# Autodesk Inventor assembly: szachy main
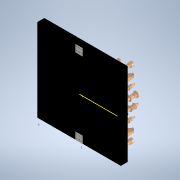
[picture p0: Inventor's stored thumbnail of the model, 180x180]
Saved by Autodesk Inventor 2021 (Build 250183000, 183)
## iProperties
Created: 2021-01-12
Part Number: szachy main
Document SubType Name: Assembly
Designer: Adam
Author: Adam
## Documents named in this file (10)
- C:\Users\Adam\Desktop\szachy main.iam
- C:\Users\Adam\Desktop\plansza 1.iam
- C:\Users\Adam\Desktop\plansza 2.iam
- C:\Users\Adam\Desktop\pret xd.ipt
- C:\Users\Adam\Desktop\goniec.ipt
- C:\Users\Adam\Desktop\król.ipt
- C:\Users\Adam\Desktop\królowa.ipt
- C:\Users\Adam\Desktop\pionek.ipt
- C:\Users\Adam\Desktop\skoczek.ipt
- C:\Users\Adam\Desktop\wieża.ipt
## Components (20 placed, 9 different names)
1. plansza 1:1 [sub-assembly] — Zestawiające:1, Zestawiające:2, Kątowe:1
2. plansza 2:1 [sub-assembly] — Zestawiające:1, Zestawiające:2, Kątowe:1, Sztywne:1, Obrotowe:1, Sztywne:2, Sztywne:3, Sztywne:4, Sztywne:5, Sztywne:6, Sztywne:7, Sztywne:8, Sztywne:9, Sztywne:10, Sztywne:11, Sztywne:12, Sztywne:13, Sztywne:14, Sztywne:15, Sztywne:16, Sztywne:17
3. pret xd:1 — Obrotowe:1
4. pret xd:2 — Sztywne:1
5. goniec:1 — Sztywne:3
6. król:1 — Sztywne:5
7. królowa:1 — Sztywne:4
8. pionek:1 — Sztywne:7
9. skoczek:1 — Sztywne:6
10. wieża:1 — Sztywne:2
11. goniec:2 — Sztywne:10
12. pionek:2 — Sztywne:11
13. skoczek:2 — Sztywne:9
14. wieża:2 — Sztywne:8
15. pionek:3 — Sztywne:16
16. pionek:4 — Sztywne:15
17. pionek:5 — Sztywne:17
18. pionek:6 — Sztywne:14
19. pionek:7 — Sztywne:12
20. pionek:8 — Sztywne:13
## Relationships (21: WeldJoint 17, Mate 2, Angle 1, RevoluteJoint 1)
- Zestawiające:1 [Mate]: plansza 1:1 ↔ plansza 2:1
- Zestawiające:2 [Mate]: plansza 1:1 ↔ plansza 2:1
- Kątowe:1 [Angle] (0 deg): plansza 1:1 ↔ plansza 2:1
- Sztywne:1 [WeldJoint]: plansza 2:1 ↔ pret xd:2
- Obrotowe:1 [RevoluteJoint]: plansza 2:1 ↔ pret xd:1
- Sztywne:2 [WeldJoint]: plansza 2:1 ↔ wieża:1
- Sztywne:3 [WeldJoint]: plansza 2:1 ↔ goniec:1
- Sztywne:4 [WeldJoint]: plansza 2:1 ↔ królowa:1
- Sztywne:5 [WeldJoint]: plansza 2:1 ↔ król:1
- Sztywne:6 [WeldJoint]: plansza 2:1 ↔ skoczek:1
- Sztywne:7 [WeldJoint]: plansza 2:1 ↔ pionek:1
- Sztywne:8 [WeldJoint]: plansza 2:1 ↔ wieża:2
- Sztywne:9 [WeldJoint]: plansza 2:1 ↔ skoczek:2
- Sztywne:10 [WeldJoint]: plansza 2:1 ↔ goniec:2
- Sztywne:11 [WeldJoint]: plansza 2:1 ↔ pionek:2
- Sztywne:12 [WeldJoint]: plansza 2:1 ↔ pionek:7
- Sztywne:13 [WeldJoint]: plansza 2:1 ↔ pionek:8
- Sztywne:14 [WeldJoint]: plansza 2:1 ↔ pionek:6
- Sztywne:15 [WeldJoint]: plansza 2:1 ↔ pionek:4
- Sztywne:16 [WeldJoint]: plansza 2:1 ↔ pionek:3
- Sztywne:17 [WeldJoint]: plansza 2:1 ↔ pionek:5
